# Autodesk Inventor assembly: 343designproper
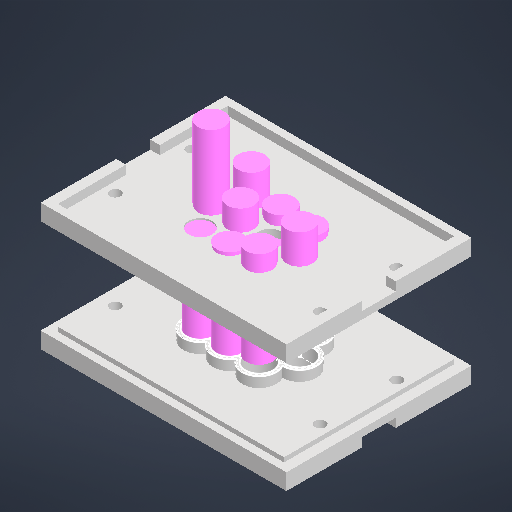
[picture p0: Inventor's stored thumbnail of the model, 512x512]
Saved by Autodesk Inventor 2025.2 (Build 292293000, 293)
## iProperties
Created: 2024-12-17
Part Number: 343designproper
Document SubType Name: Assembly
Designer: cbast
Author: cbast
## Documents named in this file (4)
- C:\Users\cbast\OneDrive\Documents\343BATTERYPACK18650.iam
- C:\Users\cbast\OneDrive\Documents\BatteryCasev1.ipt
- C:\Users\cbast\OneDrive\Documents\18650(PINK).ipt
- C:\Users\cbast\Downloads\BatteryCasev1.ipt
## Components (14 placed, 2 different names)
1. BatteryCasev1:1 — Mate:17, Mate:18
2. BatteryCasev1:2 — Mate:17, Mate:18
3. BatteryCasev1:3 — Mate:19, Mate:20, Mate:21, Mate:22, Mate:23, Mate:24, Mate:25, Mate:26, Mate:27, Mate:28
4. BatteryCasev1:4 — Mate:29, Mate:30
5. 18650(PINK):1 — Mate:19
6. 18650(PINK):2 — Mate:20
7. 18650(PINK):3 — Mate:21, Mate:30
8. 18650(PINK):4 — Mate:22
9. 18650(PINK):5 — Mate:23
10. 18650(PINK):6 — Mate:24
11. 18650(PINK):7 — Mate:25
12. 18650(PINK):8 — Mate:26, Mate:29
13. 18650(PINK):9 — Mate:27
14. 18650(PINK):10 — Mate:28
## Relationships (14: Mate 14)
- Mate:17: BatteryCasev1:1 ↔ BatteryCasev1:2
- Mate:18: BatteryCasev1:1 ↔ BatteryCasev1:2
- Mate:19: BatteryCasev1:3 ↔ 18650(PINK):1
- Mate:20: BatteryCasev1:3 ↔ 18650(PINK):2
- Mate:21: BatteryCasev1:3 ↔ 18650(PINK):3
- Mate:22: BatteryCasev1:3 ↔ 18650(PINK):4
- Mate:23: BatteryCasev1:3 ↔ 18650(PINK):5
- Mate:24: BatteryCasev1:3 ↔ 18650(PINK):6
- Mate:25: BatteryCasev1:3 ↔ 18650(PINK):7
- Mate:26: BatteryCasev1:3 ↔ 18650(PINK):8
- Mate:27: BatteryCasev1:3 ↔ 18650(PINK):9
- Mate:28: BatteryCasev1:3 ↔ 18650(PINK):10
- Mate:29: BatteryCasev1:4 ↔ 18650(PINK):8
- Mate:30: BatteryCasev1:4 ↔ 18650(PINK):3
